# Autodesk Inventor assembly: ABD_Slider_Set
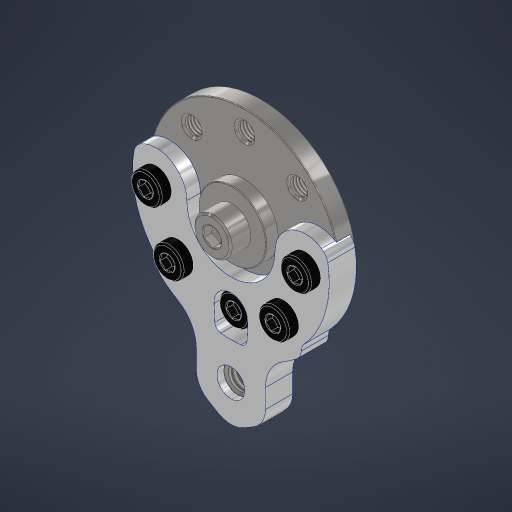
[picture p0: Inventor's stored thumbnail of the model, 512x512]
Saved by Autodesk Inventor 2024.3 (Build 283343000, 343)
## iProperties
Created: 2024-02-15
Part Number: ABD_Slider_Set
Document SubType Name: Assembly
Designer: ASUS
Author: ASUS
## Documents named in this file (6)
- C:\Users\ASUS\Desktop\Anti_Backlash_Structure_OP\v4_Frame\ABD_Slider_Set_v4.iam
- C:\Users\ASUS\Desktop\Anti_Backlash_Structure_OP\ROBOTIS(Inventor 2024 ver.)\HORN\64-106Horn.ipt
- C:\Users\ASUS\Desktop\Anti_Backlash_Structure_OP\MISUMI\CSH-STN-M3-10_203.ipt
- C:\Users\ASUS\Desktop\Anti_Backlash_Structure_OP\v4_Frame\Slider_crank_horn_v4.ipt
- C:\Users\ASUS\Documents\Inventor\Content Center Files\R2024\ko-KR\ANSI B 18.2.4.1 M(1)\ANSI B 18.2.4.1 M - M4 x 0.7Style 1.ipt
- C:\Users\ASUS\Desktop\Anti_Backlash_Structure_OP\MISUMI\CSHBTT-SUS-M2.5-4.ipt
## Components (9 placed, 5 different names)
1. 64-106Horn:1 — 삽입:3, 삽입:4, 메이트:1, 삽입:9
2. CSH-STN-M3-10_203:1 — 삽입:3
3. 6각 너트 미터 M4 x 0.7:1 — 각도:1
4. Slider_crank_horn_v3:1 — 삽입:4, 메이트:1, 삽입:5, 삽입:6, 삽입:7, 삽입:8
5. CSHBTT-SUS-M2.5-4:1 — 삽입:5
6. CSHBTT-SUS-M2.5-4:2 — 삽입:9
7. CSHBTT-SUS-M2.5-4:3 — 삽입:6
8. CSHBTT-SUS-M2.5-4:4 — 삽입:8
9. CSHBTT-SUS-M2.5-4:5 — 삽입:7
## Relationships (9: Insert 7, Angle 1, Mate 1)
- 삽입:3 [Insert]: 64-106Horn:1 ↔ CSH-STN-M3-10_203:1
- 각도:1 [Angle] (0 deg): 6각 너트 미터 M4 x 0.7:1
- 삽입:4 [Insert]: 64-106Horn:1 ↔ Slider_crank_horn_v3:1
- 메이트:1 [Mate]: 64-106Horn:1 ↔ Slider_crank_horn_v3:1
- 삽입:5 [Insert]: Slider_crank_horn_v3:1 ↔ CSHBTT-SUS-M2.5-4:1
- 삽입:6 [Insert]: Slider_crank_horn_v3:1 ↔ CSHBTT-SUS-M2.5-4:3
- 삽입:7 [Insert]: Slider_crank_horn_v3:1 ↔ CSHBTT-SUS-M2.5-4:5
- 삽입:8 [Insert]: Slider_crank_horn_v3:1 ↔ CSHBTT-SUS-M2.5-4:4
- 삽입:9 [Insert]: 64-106Horn:1 ↔ CSHBTT-SUS-M2.5-4:2
